# Autodesk Inventor assembly: LPS
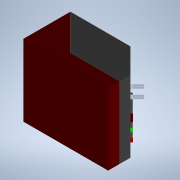
[picture p0: Inventor's stored thumbnail of the model, 180x180]
Saved by Autodesk Inventor 2022 (Build 260153000, 153)
## iProperties
Created: 2024-07-04
Part Number: LPS
Document SubType Name: Assembly
Designer: Капустяник Андрей
Author: Капустяник Андрей
## Documents named in this file (12)
- C:\Users\akapu\OneDrive\Документы\Git\camp2024\LPC_case\LPS.iam
- C:\Users\akapu\OneDrive\Документы\Git\camp2024\LPC_case\power unit.ipt
- C:\Users\akapu\OneDrive\Документы\Git\camp2024\LPC_case\LPS_board.ipt
- D:\Загрузки\User Library-potenciometro.ipt
- C:\Users\akapu\OneDrive\Документы\Git\camp2024\LPC_case\volt-amp_f2p.ipt
- C:\Users\akapu\OneDrive\Документы\Git\camp2024\LPC_case\volt-amp_f3p.ipt
- C:\Users\akapu\OneDrive\Документы\Git\camp2024\LPC_case\volt-amp_pcb.ipt
- C:\Users\akapu\OneDrive\Документы\Git\camp2024\LPC_case\volt-amp_boitier.ipt
- C:\Users\akapu\OneDrive\Документы\Git\camp2024\LPC_case\LPS_base.ipt
- C:\Users\akapu\OneDrive\Документы\Git\camp2024\LPC_case\interlock_switch_male_wFuse v13.ipt
- C:\Users\akapu\OneDrive\Документы\Git\camp2024\LPC_case\LPS_cap.ipt
- C:\Users\akapu\OneDrive\Документы\Git\camp2024\LPC_case\User Library-fan_5010.ipt
## Components (12 placed, 11 different names)
1. power unit:1 — Заподлицо:1
2. LPS_board:1
3. User Library-potenciometro:2 — Совмещение:13
4. User Library-potenciometro:3 — Совмещение:12
5. volt-amp_f2p:1 — Совмещение:1, Совмещение:2, Совмещение:3
6. volt-amp_f3p:1 — Совмещение:4, Совмещение:5, Совмещение:6
7. volt-amp_pcb:1 — Совмещение:1, Совмещение:2, Совмещение:3, Совмещение:4, Совмещение:5, Совмещение:6, Совмещение:7, Совмещение:8, Совмещение:9
8. volt-amp_boitier:1 — Совмещение:7, Совмещение:8, Совмещение:9, Совмещение:11
9. LPS_base:1 — Заподлицо:1, Совмещение:10, Заподлицо:2
10. interlock_switch_male_wFuse v13:1 — Совмещение:10
11. LPS_cap:1 — Заподлицо:2, Совмещение:11, Совмещение:12, Совмещение:13, Совмещение:14, Совмещение:15
12. User Library-fan_5010:1 — Совмещение:14, Совмещение:15
## Relationships (17: Mate 15, Flush 2)
- Совмещение:1 [Mate]: volt-amp_f2p:1 ↔ volt-amp_pcb:1
- Совмещение:2 [Mate]: volt-amp_f2p:1 ↔ volt-amp_pcb:1
- Совмещение:3 [Mate]: volt-amp_f2p:1 ↔ volt-amp_pcb:1
- Совмещение:4 [Mate]: volt-amp_f3p:1 ↔ volt-amp_pcb:1
- Совмещение:5 [Mate]: volt-amp_f3p:1 ↔ volt-amp_pcb:1
- Совмещение:6 [Mate]: volt-amp_f3p:1 ↔ volt-amp_pcb:1
- Совмещение:7 [Mate]: volt-amp_pcb:1 ↔ volt-amp_boitier:1
- Совмещение:8 [Mate]: volt-amp_pcb:1 ↔ volt-amp_boitier:1
- Совмещение:9 [Mate]: volt-amp_pcb:1 ↔ volt-amp_boitier:1
- Заподлицо:1 [Flush]: power unit:1 ↔ LPS_base:1
- Совмещение:10 [Mate]: LPS_base:1 ↔ interlock_switch_male_wFuse v13:1
- Заподлицо:2 [Flush]: LPS_base:1 ↔ LPS_cap:1
- Совмещение:11 [Mate]: volt-amp_boitier:1 ↔ LPS_cap:1
- Совмещение:12 [Mate]: User Library-potenciometro:3 ↔ LPS_cap:1
- Совмещение:13 [Mate]: User Library-potenciometro:2 ↔ LPS_cap:1
- Совмещение:14 [Mate]: LPS_cap:1 ↔ User Library-fan_5010:1
- Совмещение:15 [Mate]: LPS_cap:1 ↔ User Library-fan_5010:1
